# Autodesk Inventor assembly: New Box ARm
(part 2 of 2)
- Mate:204: Clamping_Shaft_Collar_-_1_2_Hex_ID_217-2737:1 ↔ Hex Shaft ARm:1
- Mate:205: Clamping_Shaft_Collar_-_1_2_Hex_ID_217-2737:1 ↔ Hex Shaft ARm:1
- Mate:213: 1_2_Acetal_Spacer_-_1_2_Hex_217-3261:1 ↔ Hex Shaft ARm:1
- Mate:214: 1_2_Acetal_Spacer_-_1_2_Hex_217-3261:1 ↔ Hex Shaft ARm:1
- Mate:215: 1_2_Acetal_Spacer_-_1_2_Hex_217-3261:1 ↔ 0_500_ID_x_1_125_OD_x_0_313_WD_Flanged_Bearing_217-2731:2
- Mate:222: 41.75in Arm Beam Alternate (Right):1 ↔ Hex Hub:2
- Mate:224: Hex Hub:2 ↔ Hex Shaft ARm:1
- Mate:225: Hex Hub:2 ↔ Hex Shaft ARm:1
- Mate:230: Hex Shaft ARm:1 ↔ 1_2_Acetal_Spacer_-_1_2_Hex_217-3261:4
- Mate:231: Hex Shaft ARm:1 ↔ 1_2_Acetal_Spacer_-_1_2_Hex_217-3261:4
- Mate:232: 1_2_Acetal_Spacer_-_1_2_Hex_217-3261:4 ↔ 0_500_ID_x_1_125_OD_x_0_313_WD_Flanged_Bearing_217-2731:3
- Mate:236: Hex Shaft ARm:1 ↔ Clamping_Shaft_Collar_-_1_2_Hex_ID_217-2737:2
- Mate:237: Hex Shaft ARm:1 ↔ Clamping_Shaft_Collar_-_1_2_Hex_ID_217-2737:2
- Mate:240: Hex Shaft ARm:1 ↔ Hex Hub:3
- Mate:241: Hex Shaft ARm:1 ↔ Hex Hub:3
- Rotation:2 [RelateRotation] (1 ul): Hex Shaft ARm:1 ↔ Hex Hub:3
- Rotation:4 [RelateRotation] (1 ul): Hex Hub:2 ↔ Hex Shaft ARm:1
- Mate:242: 15in Horizontal 1x1 Beam:1 ↔ 41.75in Arm Beam Alternate (Right):1
- Mate:259: L gusset:9 ↔ 1.5in 92196A251_18-8 STAINLESS STEEL SOCKET HEAD CAP SCREW:13
- Mate:260: L gusset:9 ↔ 1.5in 92196A251_18-8 STAINLESS STEEL SOCKET HEAD CAP SCREW:39
- Mate:261: L gusset:9 ↔ 1.5in 92196A251_18-8 STAINLESS STEEL SOCKET HEAD CAP SCREW:24
- Mate:263: L gusset:9 ↔ 1.5in 92196A251_18-8 STAINLESS STEEL SOCKET HEAD CAP SCREW:38
- Mate:268: L gusset:14 ↔ 1.5in 92196A251_18-8 STAINLESS STEEL SOCKET HEAD CAP SCREW:49
- Mate:269: L gusset:14 ↔ 1.5in 92196A251_18-8 STAINLESS STEEL SOCKET HEAD CAP SCREW:47
- Mate:270: L gusset:14 ↔ 1.5in 92196A251_18-8 STAINLESS STEEL SOCKET HEAD CAP SCREW:10
- Mate:271: L gusset:14 ↔ 1.5in 92196A251_18-8 STAINLESS STEEL SOCKET HEAD CAP SCREW:9
- Mate:272: L gusset:14 ↔ 1.5in 92196A251_18-8 STAINLESS STEEL SOCKET HEAD CAP SCREW:45
- Mate:273: L gusset:8 ↔ 1.5in 92196A251_18-8 STAINLESS STEEL SOCKET HEAD CAP SCREW:35
- Mate:274: L gusset:8 ↔ 1.5in 92196A251_18-8 STAINLESS STEEL SOCKET HEAD CAP SCREW:36
- Mate:275: L gusset:8 ↔ 1.5in 92196A251_18-8 STAINLESS STEEL SOCKET HEAD CAP SCREW:25
- Mate:277: L gusset:8 ↔ 1.5in 92196A251_18-8 STAINLESS STEEL SOCKET HEAD CAP SCREW:43
- Mate:278: L gusset:14 ↔ 1.5in 92196A251_18-8 STAINLESS STEEL SOCKET HEAD CAP SCREW:47
- Mate:279: L gusset:14 ↔ 1.5in 92196A251_18-8 STAINLESS STEEL SOCKET HEAD CAP SCREW:49
- Mate:280: L gusset:14 ↔ 1.5in 92196A251_18-8 STAINLESS STEEL SOCKET HEAD CAP SCREW:10
- Mate:281: L gusset:14 ↔ 1.5in 92196A251_18-8 STAINLESS STEEL SOCKET HEAD CAP SCREW:9
- Mate:282: L gusset:14 ↔ 1.5in 92196A251_18-8 STAINLESS STEEL SOCKET HEAD CAP SCREW:45
- Mate:285: L gusset:9 ↔ 1.5in 92196A251_18-8 STAINLESS STEEL SOCKET HEAD CAP SCREW:39
- Mate:286: L gusset:9 ↔ 1.5in 92196A251_18-8 STAINLESS STEEL SOCKET HEAD CAP SCREW:24
- Mate:287: L gusset:9 ↔ 1.5in 92196A251_18-8 STAINLESS STEEL SOCKET HEAD CAP SCREW:38
- Mate:288: L gusset:9 ↔ 1.5in 92196A251_18-8 STAINLESS STEEL SOCKET HEAD CAP SCREW:13
- Mate:289: L gusset:8 ↔ 1.5in 92196A251_18-8 STAINLESS STEEL SOCKET HEAD CAP SCREW:43
- Mate:291: L gusset:8 ↔ 1.5in 92196A251_18-8 STAINLESS STEEL SOCKET HEAD CAP SCREW:25
- Mate:292: L gusset:8 ↔ 1.5in 92196A251_18-8 STAINLESS STEEL SOCKET HEAD CAP SCREW:36
- Mate:293: L gusset:8 ↔ 1.5in 92196A251_18-8 STAINLESS STEEL SOCKET HEAD CAP SCREW:35
- Mate:296: L gusset:10 ↔ 1.5in 92196A251_18-8 STAINLESS STEEL SOCKET HEAD CAP SCREW:34
- Mate:297: L gusset:10 ↔ 1.5in 92196A251_18-8 STAINLESS STEEL SOCKET HEAD CAP SCREW:15
- Mate:298: L gusset:10 ↔ 1.5in 92196A251_18-8 STAINLESS STEEL SOCKET HEAD CAP SCREW:17
- Mate:300: 24in Vertical 1x1 Beam:3 ↔ LV Gusset:2
- Mate:301: 25in Horizontal 1x1 Beam:1 ↔ LV Gusset:2
- Mate:302: 25in Horizontal 1x1 Beam:1 ↔ LV Gusset:2
- Mate:303: 25in Horizontal 1x1 Beam:1 ↔ LV Gusset:2
- Mate:304: 24in Vertical 1x1 Beam:3 ↔ LV Gusset:2
- Mate:305: 24in Vertical 1x1 Beam:3 ↔ LV Gusset:2
- Mate:306: 24in Vertical 1x1 Beam:4 ↔ LV Gusset:1
- Mate:307: 25in Horizontal 1x1 Beam:2 ↔ LV Gusset:1
- Mate:308: 25in Horizontal 1x1 Beam:2 ↔ LV Gusset:1
- Mate:309: 25in Horizontal 1x1 Beam:2 ↔ LV Gusset:1
- Mate:310: 24in Vertical 1x1 Beam:4 ↔ LV Gusset:1
- Mate:311: 24in Vertical 1x1 Beam:4 ↔ LV Gusset:1
- Flush:129: 25in Horizontal 1x1 Beam:2 ↔ LV Gusset:1
- Flush:130: 24in Vertical 1x1 Beam:4 ↔ LV Gusset:1
- Flush:131: 24in Vertical 1x1 Beam:4 ↔ LV Gusset:1
- Flush:132: 25in Horizontal 1x1 Beam:2 ↔ LV Gusset:1
- Flush:133: 25in Horizontal 1x1 Beam:1 ↔ LV Gusset:2
- Flush:134: 24in Vertical 1x1 Beam:3 ↔ LV Gusset:2
- Flush:135: 24in Vertical 1x1 Beam:3 ↔ LV Gusset:2
- Flush:136: 25in Horizontal 1x1 Beam:1 ↔ LV Gusset:2
- Mate:312: 1.5in 92196A251_18-8 STAINLESS STEEL SOCKET HEAD CAP SCREW:7 ↔ LV Gusset:2
- Mate:313: 1.5in 92196A251_18-8 STAINLESS STEEL SOCKET HEAD CAP SCREW:11 ↔ LV Gusset:2
- Mate:314: 1.5in 92196A251_18-8 STAINLESS STEEL SOCKET HEAD CAP SCREW:11 ↔ LV Gusset:2
- Mate:315: 1.5in 92196A251_18-8 STAINLESS STEEL SOCKET HEAD CAP SCREW:7 ↔ LV Gusset:2
- Mate:316: 1.5in 92196A251_18-8 STAINLESS STEEL SOCKET HEAD CAP SCREW:14 ↔ LV Gusset:2
- Mate:317: 1.5in 92196A251_18-8 STAINLESS STEEL SOCKET HEAD CAP SCREW:2 ↔ LV Gusset:2
- Mate:318: 1.5in 92196A251_18-8 STAINLESS STEEL SOCKET HEAD CAP SCREW:14 ↔ LV Gusset:2
- Mate:319: 1.5in 92196A251_18-8 STAINLESS STEEL SOCKET HEAD CAP SCREW:2 ↔ LV Gusset:2
- Mate:320: 1.5in 92196A251_18-8 STAINLESS STEEL SOCKET HEAD CAP SCREW:1 ↔ LV Gusset:1
- Mate:321: 1.5in 92196A251_18-8 STAINLESS STEEL SOCKET HEAD CAP SCREW:20 ↔ LV Gusset:1
- Mate:322: 1.5in 92196A251_18-8 STAINLESS STEEL SOCKET HEAD CAP SCREW:1 ↔ LV Gusset:1
- Mate:323: 1.5in 92196A251_18-8 STAINLESS STEEL SOCKET HEAD CAP SCREW:20 ↔ LV Gusset:1
- Mate:324: 1.5in 92196A251_18-8 STAINLESS STEEL SOCKET HEAD CAP SCREW:3 ↔ LV Gusset:1
- Mate:325: 1.5in 92196A251_18-8 STAINLESS STEEL SOCKET HEAD CAP SCREW:8 ↔ LV Gusset:1
- Mate:326: 1.5in 92196A251_18-8 STAINLESS STEEL SOCKET HEAD CAP SCREW:8 ↔ LV Gusset:1
- Mate:327: 1.5in 92196A251_18-8 STAINLESS STEEL SOCKET HEAD CAP SCREW:3 ↔ LV Gusset:1
- Mate:328: L gusset:10 ↔ 1.5in 92196A251_18-8 STAINLESS STEEL SOCKET HEAD CAP SCREW:34
- Mate:329: L gusset:10 ↔ 1.5in 92196A251_18-8 STAINLESS STEEL SOCKET HEAD CAP SCREW:15
- Mate:330: L gusset:10 ↔ 1.5in 92196A251_18-8 STAINLESS STEEL SOCKET HEAD CAP SCREW:17
- Mate:332: L gusset:13 ↔ 1.5in 92196A251_18-8 STAINLESS STEEL SOCKET HEAD CAP SCREW:12
- Mate:333: L gusset:13 ↔ 1.5in 92196A251_18-8 STAINLESS STEEL SOCKET HEAD CAP SCREW:26
- Mate:334: L gusset:13 ↔ 1.5in 92196A251_18-8 STAINLESS STEEL SOCKET HEAD CAP SCREW:22
- Mate:335: L gusset:13 ↔ 1.5in 92196A251_18-8 STAINLESS STEEL SOCKET HEAD CAP SCREW:30
- Mate:336: L gusset:13 ↔ 1.5in 92196A251_18-8 STAINLESS STEEL SOCKET HEAD CAP SCREW:18
- Mate:337: L gusset:10 ↔ 1.5in 92196A251_18-8 STAINLESS STEEL SOCKET HEAD CAP SCREW:28
- Mate:338: L gusset:10 ↔ 1.5in 92196A251_18-8 STAINLESS STEEL SOCKET HEAD CAP SCREW:28
- Mate:339: L gusset:15 ↔ 1.5in 92196A251_18-8 STAINLESS STEEL SOCKET HEAD CAP SCREW:21
- Mate:340: L gusset:15 ↔ 1.5in 92196A251_18-8 STAINLESS STEEL SOCKET HEAD CAP SCREW:21
- Mate:341: L gusset:15 ↔ 1.5in 92196A251_18-8 STAINLESS STEEL SOCKET HEAD CAP SCREW:5
- Mate:342: L gusset:15 ↔ 1.5in 92196A251_18-8 STAINLESS STEEL SOCKET HEAD CAP SCREW:52
- Mate:343: L gusset:19 ↔ 1.5in 92196A251_18-8 STAINLESS STEEL SOCKET HEAD CAP SCREW:51
- Mate:344: L gusset:19 ↔ 1.5in 92196A251_18-8 STAINLESS STEEL SOCKET HEAD CAP SCREW:58
- Mate:345: L gusset:19 ↔ 1.5in 92196A251_18-8 STAINLESS STEEL SOCKET HEAD CAP SCREW:59
- Mate:346: L gusset:19 ↔ 1.5in 92196A251_18-8 STAINLESS STEEL SOCKET HEAD CAP SCREW:59
- Mate:347: L gusset:19 ↔ 1.5in 92196A251_18-8 STAINLESS STEEL SOCKET HEAD CAP SCREW:58
- Mate:348: L gusset:19 ↔ 1.5in 92196A251_18-8 STAINLESS STEEL SOCKET HEAD CAP SCREW:51
- Mate:349: L gusset:15 ↔ 1.5in 92196A251_18-8 STAINLESS STEEL SOCKET HEAD CAP SCREW:52
- Mate:350: L gusset:15 ↔ 1.5in 92196A251_18-8 STAINLESS STEEL SOCKET HEAD CAP SCREW:5
- Mate:351: L gusset:16 ↔ 1.5in 92196A251_18-8 STAINLESS STEEL SOCKET HEAD CAP SCREW:67
- Mate:352: L gusset:16 ↔ 1.5in 92196A251_18-8 STAINLESS STEEL SOCKET HEAD CAP SCREW:61
- Mate:353: L gusset:18 ↔ 1.5in 92196A251_18-8 STAINLESS STEEL SOCKET HEAD CAP SCREW:64
- Mate:354: L gusset:18 ↔ 1.5in 92196A251_18-8 STAINLESS STEEL SOCKET HEAD CAP SCREW:60
- Mate:355: L gusset:18 ↔ 1.5in 92196A251_18-8 STAINLESS STEEL SOCKET HEAD CAP SCREW:60
- Mate:356: L gusset:18 ↔ 1.5in 92196A251_18-8 STAINLESS STEEL SOCKET HEAD CAP SCREW:64
- Mate:357: L gusset:16 ↔ 1.5in 92196A251_18-8 STAINLESS STEEL SOCKET HEAD CAP SCREW:67
- Mate:358: L gusset:16 ↔ 1.5in 92196A251_18-8 STAINLESS STEEL SOCKET HEAD CAP SCREW:61
- Mate:359: L gusset:13 ↔ 1.5in 92196A251_18-8 STAINLESS STEEL SOCKET HEAD CAP SCREW:22
- Mate:360: L gusset:13 ↔ 1.5in 92196A251_18-8 STAINLESS STEEL SOCKET HEAD CAP SCREW:26
- Mate:361: L gusset:13 ↔ 1.5in 92196A251_18-8 STAINLESS STEEL SOCKET HEAD CAP SCREW:12
- Mate:362: L gusset:13 ↔ 1.5in 92196A251_18-8 STAINLESS STEEL SOCKET HEAD CAP SCREW:30
- Mate:363: L gusset:13 ↔ 1.5in 92196A251_18-8 STAINLESS STEEL SOCKET HEAD CAP SCREW:18
- Mate:364: L gusset:11 ↔ 1.5in 92196A251_18-8 STAINLESS STEEL SOCKET HEAD CAP SCREW:6
- Mate:365: L gusset:11 ↔ 1.5in 92196A251_18-8 STAINLESS STEEL SOCKET HEAD CAP SCREW:27
- Mate:366: L gusset:11 ↔ 1.5in 92196A251_18-8 STAINLESS STEEL SOCKET HEAD CAP SCREW:19
- Mate:368: L gusset:11 ↔ 1.5in 92196A251_18-8 STAINLESS STEEL SOCKET HEAD CAP SCREW:31
- Mate:369: L gusset:11 ↔ 1.5in 92196A251_18-8 STAINLESS STEEL SOCKET HEAD CAP SCREW:6
- Mate:370: L gusset:11 ↔ 1.5in 92196A251_18-8 STAINLESS STEEL SOCKET HEAD CAP SCREW:27
- Mate:372: L gusset:11 ↔ 1.5in 92196A251_18-8 STAINLESS STEEL SOCKET HEAD CAP SCREW:19
- Mate:373: L gusset:11 ↔ 1.5in 92196A251_18-8 STAINLESS STEEL SOCKET HEAD CAP SCREW:31
- Mate:376: L gusset:17 ↔ .75in 92196A245_18-8 STAINLESS STEEL SOCKET HEAD CAP SCREW:1
- Mate:377: L gusset:17 ↔ .75in 92196A245_18-8 STAINLESS STEEL SOCKET HEAD CAP SCREW:1
- Mate:380: L gusset:11 ↔ 1.5in 92196A251_18-8 STAINLESS STEEL SOCKET HEAD CAP SCREW:68
- Mate:381: L gusset:11 ↔ 1.5in 92196A251_18-8 STAINLESS STEEL SOCKET HEAD CAP SCREW:68
- Mate:382: L gusset:8 ↔ 1.5in 92196A251_18-8 STAINLESS STEEL SOCKET HEAD CAP SCREW:69
- Mate:383: L gusset:8 ↔ 1.5in 92196A251_18-8 STAINLESS STEEL SOCKET HEAD CAP SCREW:69
- Mate:384: L gusset:20 ↔ .75in 92196A245_18-8 STAINLESS STEEL SOCKET HEAD CAP SCREW:34
- Mate:385: L gusset:20 ↔ .75in 92196A245_18-8 STAINLESS STEEL SOCKET HEAD CAP SCREW:34
- Mate:386: L gusset:20 ↔ .75in 92196A245_18-8 STAINLESS STEEL SOCKET HEAD CAP SCREW:14
- Mate:387: L gusset:20 ↔ .75in 92196A245_18-8 STAINLESS STEEL SOCKET HEAD CAP SCREW:15
- Mate:388: L gusset:17 ↔ .75in 92196A245_18-8 STAINLESS STEEL SOCKET HEAD CAP SCREW:17
- Mate:389: L gusset:17 ↔ .75in 92196A245_18-8 STAINLESS STEEL SOCKET HEAD CAP SCREW:58
- Mate:390: L gusset:17 ↔ .75in 92196A245_18-8 STAINLESS STEEL SOCKET HEAD CAP SCREW:17
- Mate:391: L gusset:17 ↔ .75in 92196A245_18-8 STAINLESS STEEL SOCKET HEAD CAP SCREW:58
- Mate:392: L gusset:20 ↔ .75in 92196A245_18-8 STAINLESS STEEL SOCKET HEAD CAP SCREW:14
- Mate:393: L gusset:20 ↔ .75in 92196A245_18-8 STAINLESS STEEL SOCKET HEAD CAP SCREW:15
- Mate:394: L gusset:17 ↔ 1.5in 92196A251_18-8 STAINLESS STEEL SOCKET HEAD CAP SCREW:54
- Mate:395: L gusset:17 ↔ 1.5in 92196A251_18-8 STAINLESS STEEL SOCKET HEAD CAP SCREW:33
- Mate:396: L gusset:20 ↔ 1.5in 92196A251_18-8 STAINLESS STEEL SOCKET HEAD CAP SCREW:56
- Mate:397: L gusset:20 ↔ 1.5in 92196A251_18-8 STAINLESS STEEL SOCKET HEAD CAP SCREW:50
- Mate:398: L gusset:20 ↔ 1.5in 92196A251_18-8 STAINLESS STEEL SOCKET HEAD CAP SCREW:56
- Mate:399: L gusset:20 ↔ 1.5in 92196A251_18-8 STAINLESS STEEL SOCKET HEAD CAP SCREW:50
- Mate:400: L gusset:17 ↔ 1.5in 92196A251_18-8 STAINLESS STEEL SOCKET HEAD CAP SCREW:54
- Mate:401: L gusset:17 ↔ 1.5in 92196A251_18-8 STAINLESS STEEL SOCKET HEAD CAP SCREW:33
- Mate:403: 41.75in Arm Beam Alternate (Right):1 ↔ 0_500_ID_x_1_125_OD_x_0_313_WD_Flanged_Bearing_217-2731:6
- Mate:404: 41.75in Arm Beam Alternate (Right):1 ↔ 0_500_ID_x_1_125_OD_x_0_313_WD_Flanged_Bearing_217-2731:7
- Mate:409: 41.75in Arm Beam Alternate (Right):1 ↔ 0_500_ID_x_1_125_OD_x_0_313_WD_Flanged_Bearing_217-2731:6
- Mate:410: 41.75in Arm Beam Alternate (Right):1 ↔ 0_500_ID_x_1_125_OD_x_0_313_WD_Flanged_Bearing_217-2731:7
- Mate:411: 41.75in Arm Beam Alternate (Right):1 ↔ 0_500_Hex_ID_x_1_125_OD_x_0_313_WD_Flanged_Bearing_v2_217-3875:1
- Mate:418: 41.75in Arm Beam Alternate (Right):1 ↔ 0_500_Hex_ID_x_1_125_OD_x_0_313_WD_Flanged_Bearing_v2_217-3875:1
- Mate:419: 41.75in Arm Beam Alternate (Right):1 ↔ VersaPlanetary_v2_Two_Stage_100_1_with_BAG:1
- Mate:420: 41.75in Arm Beam Alternate (Right):1 ↔ VersaPlanetary_v2_Two_Stage_100_1_with_BAG:1
- Mate:421: 41.75in Arm Beam Alternate (Right):1 ↔ VersaPlanetary_v2_Two_Stage_100_1_with_BAG:1
- Mate:422: am-3621 - S25-18HA-500H:1 ↔ VersaPlanetary_v2_Two_Stage_100_1_with_BAG:1
- Mate:423: am-3621 - S25-18HA-500H:1 ↔ VersaPlanetary_v2_Two_Stage_100_1_with_BAG:1
- Mate:424: am-3621 - S25-18HA-500H:1 ↔ 0_500_Hex_ID_x_1_125_OD_x_0_313_WD_Flanged_Bearing_v2_217-3875:1
- Mate:426: VersaPlanetary_v2_Two_Stage_100_1_with_BAG:1 ↔ 3D Model Spacer Arm:1
- Mate:427: VersaPlanetary_v2_Two_Stage_100_1_with_BAG:1 ↔ 3D Model Spacer Arm:1
- Mate:428: am-3621 - S25-18HA-500H:1 ↔ 3D Model Spacer Arm:1
- Mate:429: VersaPlanetary_v2_Two_Stage_100_1_with_BAG:1 ↔ 92240A537_18-8 STAINLESS STEEL HEX HEAD CAP SCREW:1
- Mate:430: 92240A537_18-8 STAINLESS STEEL HEX HEAD CAP SCREW:1 ↔ 3D Model Washer Arm Gearbo:1
- Mate:431: 3D Model Spacer Arm:1 ↔ 3D Model Washer Arm Gearbo:1
- Mate:432: 92240A537_18-8 STAINLESS STEEL HEX HEAD CAP SCREW:1 ↔ 3D Model Washer Arm Gearbo:1
- Mate:437: Wrist Hex Shaft 0.5in:1 ↔ Clamping_Shaft_Collar_-_1_2_Hex_ID_217-2737:6
- Mate:438: Wrist Hex Shaft 0.5in:1 ↔ Clamping_Shaft_Collar_-_1_2_Hex_ID_217-2737:6
- Flush:138: Wrist Hex Shaft 0.5in:1 ↔ Clamping_Shaft_Collar_-_1_2_Hex_ID_217-2737:6
- Mate:439: Wrist Hex Shaft 0.5in:1 ↔ Clamping_Shaft_Collar_-_1_2_Hex_ID_217-2737:5
- Mate:440: Wrist Hex Shaft 0.5in:1 ↔ Clamping_Shaft_Collar_-_1_2_Hex_ID_217-2737:5
- Mate:441: Wrist Hex Shaft 0.5in:1 ↔ Clamping_Shaft_Collar_-_1_2_Hex_ID_217-2737:4
- Mate:442: Wrist Hex Shaft 0.5in:1 ↔ Clamping_Shaft_Collar_-_1_2_Hex_ID_217-2737:4
- Mate:443: Wrist Hex Shaft 0.5in:1 ↔ 1_16_Acetal_Spacer_-_1_2_Hex_217-3257:2
- Mate:444: Wrist Hex Shaft 0.5in:1 ↔ 1_16_Acetal_Spacer_-_1_2_Hex_217-3257:2
- Mate:445: Wrist Hex Shaft 0.5in:1 ↔ 1_16_Acetal_Spacer_-_1_2_Hex_217-3257:1
- Mate:446: Wrist Hex Shaft 0.5in:1 ↔ 1_16_Acetal_Spacer_-_1_2_Hex_217-3257:1
- Mate:447: 0_500_ID_x_1_125_OD_x_0_313_WD_Flanged_Bearing_217-2731:6 ↔ 1_16_Acetal_Spacer_-_1_2_Hex_217-3257:1
- Mate:448: Clamping_Shaft_Collar_-_1_2_Hex_ID_217-2737:4 ↔ 1_16_Acetal_Spacer_-_1_2_Hex_217-3257:1
- Mate:449: 0_500_ID_x_1_125_OD_x_0_313_WD_Flanged_Bearing_217-2731:5 ↔ 1_16_Acetal_Spacer_-_1_2_Hex_217-3257:2
- Mate:450: Clamping_Shaft_Collar_-_1_2_Hex_ID_217-2737:5 ↔ 1_16_Acetal_Spacer_-_1_2_Hex_217-3257:2
- Mate:451: am-3621 - S25-18HA-500H:2 ↔ Wrist Hex Shaft 0.5in:1
- Mate:452: am-3621 - S25-18HA-500H:2 ↔ Wrist Hex Shaft 0.5in:1
- Mate:453: 0_500_ID_x_1_125_OD_x_0_313_WD_Flanged_Bearing_217-2731:7 ↔ am-3621 - S25-18HA-500H:2
- Flush:140: am-3621 - S25-18HA-500H:1 ↔ am-3621 - S25-18HA-500H:2
- Mate:459: 0_500_ID_x_1_125_OD_x_0_313_WD_Flanged_Bearing_217-2731:6 ↔ 1_16_Acetal_Spacer_-_1_2_Hex_217-3257:1
- Mate:460: 0_500_ID_x_1_125_OD_x_0_313_WD_Flanged_Bearing_217-2731:8 ↔ Clamping_Shaft_Collar_-_1_2_Hex_ID_217-2737:6
- Mate:482: Hex Hub:3 ↔ 41.75in Arm Beam Alternate (Left):1
- Mate:488: Hex Hub:3 ↔ 41.75in Arm Beam Alternate (Left):1
- Mate:489: 0_500_ID_x_1_125_OD_x_0_313_WD_Flanged_Bearing_217-2731:10 ↔ 41.75in Arm Beam Alternate (Left):1
- Mate:490: 0_500_ID_x_1_125_OD_x_0_313_WD_Flanged_Bearing_217-2731:10 ↔ 41.75in Arm Beam Alternate (Left):1
- Mate:491: 41.75in Arm Beam Alternate (Right):1 ↔ 0_500_ID_x_1_125_OD_x_0_313_WD_Flanged_Bearing_217-2731:9
- Mate:492: 41.75in Arm Beam Alternate (Right):1 ↔ 0_500_ID_x_1_125_OD_x_0_313_WD_Flanged_Bearing_217-2731:9
- Mate:493: 0_500_ID_x_1_125_OD_x_0_313_WD_Flanged_Bearing_217-2731:8 ↔ Clamping_Shaft_Collar_-_1_2_Hex_ID_217-2737:6
- Mate:494: 0_500_ID_x_1_125_OD_x_0_313_WD_Flanged_Bearing_217-2731:5 ↔ 41.75in Arm Beam Alternate (Left):1
- Mate:495: 0_500_ID_x_1_125_OD_x_0_313_WD_Flanged_Bearing_217-2731:5 ↔ 41.75in Arm Beam Alternate (Left):1
- Mate:506: 15in Horizontal 1x1 Beam:2 ↔ 1x1 Bumper Attachment:2
- Mate:507: 15in Horizontal 1x1 Beam:2 ↔ 1x1 Bumper Attachment:2
- Mate:508: 15in Horizontal 1x1 Beam:2 ↔ 1x1 Bumper Attachment:2
- Mate:509: 15in Horizontal 1x1 Beam:1 ↔ 1x1 Bumper Attachment:1
- Mate:510: 15in Horizontal 1x1 Beam:1 ↔ 1x1 Bumper Attachment:1
- Mate:511: 15in Horizontal 1x1 Beam:1 ↔ 1x1 Bumper Attachment:1
- Mate:512: 1x1 Bumper Attachment:2 ↔ 042:1
- Mate:513: 1x1 Bumper Attachment:2 ↔ 042:1
- Mate:514: 1x1 Bumper Attachment:1 ↔ 042:2
- Mate:515: 1x1 Bumper Attachment:1 ↔ 042:2
- Mate:516: 15in Horizontal 1x1 Beam:1 ↔ Arm Belly Pan:1
- Mate:517: L gusset:1 ↔ Arm Belly Pan:1
- Flush:141: 15in Horizontal 1x1 Beam:1 ↔ Arm Belly Pan:1
- Mate:518: Hex Hub:3 ↔ 41.75in Arm Beam Alternate (Left):1
- Mate:519: Hex Hub:3 ↔ 41.75in Arm Beam Alternate (Left):1
- Mate:522: Arm Belly Pan:1 ↔ 73434-Fastenal-01-12-2019:2
- Mate:523: Arm Belly Pan:1 ↔ 73434-Fastenal-01-12-2019:1
- Mate:524: Arm Belly Pan:1 ↔ 73434-Fastenal-01-12-2019:2
- Mate:525: Arm Belly Pan:1 ↔ 73434-Fastenal-01-12-2019:1
- Mate:526: Arm Belly Pan:1 ↔ 73434-Fastenal-01-12-2019:4
- Mate:527: Arm Belly Pan:1 ↔ 73434-Fastenal-01-12-2019:3
- Mate:528: Arm Belly Pan:1 ↔ 73434-Fastenal-01-12-2019:3
- Mate:529: Arm Belly Pan:1 ↔ 73434-Fastenal-01-12-2019:4
- Mate:530: 1x1 Bumper Attachment:1 ↔ 91831A011_TYPE 18-8 STAINLESS STL NYLON-INSERT LOCKNUT:4
- Mate:531: 73434-Fastenal-01-12-2019:3 ↔ 91831A011_TYPE 18-8 STAINLESS STL NYLON-INSERT LOCKNUT:4
- Mate:532: 1x1 Bumper Attachment:1 ↔ 91831A011_TYPE 18-8 STAINLESS STL NYLON-INSERT LOCKNUT:3
- Mate:533: 73434-Fastenal-01-12-2019:4 ↔ 91831A011_TYPE 18-8 STAINLESS STL NYLON-INSERT LOCKNUT:3
- Mate:534: 1x1 Bumper Attachment:2 ↔ 91831A011_TYPE 18-8 STAINLESS STL NYLON-INSERT LOCKNUT:2
- Mate:535: 73434-Fastenal-01-12-2019:1 ↔ 91831A011_TYPE 18-8 STAINLESS STL NYLON-INSERT LOCKNUT:2
- Mate:536: 1x1 Bumper Attachment:2 ↔ 91831A011_TYPE 18-8 STAINLESS STL NYLON-INSERT LOCKNUT:1
- Mate:537: 73434-Fastenal-01-12-2019:2 ↔ 91831A011_TYPE 18-8 STAINLESS STL NYLON-INSERT LOCKNUT:1
- Mate:538: Arm Belly Pan:1 ↔ 1.5in 92196A251_18-8 STAINLESS STEEL SOCKET HEAD CAP SCREW:73
- Mate:539: Arm Belly Pan:1 ↔ 1.5in 92196A251_18-8 STAINLESS STEEL SOCKET HEAD CAP SCREW:72
- Mate:540: Arm Belly Pan:1 ↔ 1.5in 92196A251_18-8 STAINLESS STEEL SOCKET HEAD CAP SCREW:70
- Mate:541: Arm Belly Pan:1 ↔ 1.5in 92196A251_18-8 STAINLESS STEEL SOCKET HEAD CAP SCREW:71
- Mate:542: Arm Belly Pan:1 ↔ 73434-Fastenal-01-12-2019:6
- Mate:543: Arm Belly Pan:1 ↔ 73434-Fastenal-01-12-2019:5
- Mate:544: Arm Belly Pan:1 ↔ 73434-Fastenal-01-12-2019:8
- Mate:545: Arm Belly Pan:1 ↔ 73434-Fastenal-01-12-2019:7
- Mate:546 (3.175 mm): Arm Belly Pan:1 ↔ 73434-Fastenal-01-12-2019:7
- Mate:547 (3.175 mm): Arm Belly Pan:1 ↔ 73434-Fastenal-01-12-2019:8
- Mate:548 (3.175 mm): Arm Belly Pan:1 ↔ 1.5in 92196A251_18-8 STAINLESS STEEL SOCKET HEAD CAP SCREW:73
- Mate:549 (3.175 mm): Arm Belly Pan:1 ↔ 1.5in 92196A251_18-8 STAINLESS STEEL SOCKET HEAD CAP SCREW:72
- Mate:550 (3.175 mm): Arm Belly Pan:1 ↔ 1.5in 92196A251_18-8 STAINLESS STEEL SOCKET HEAD CAP SCREW:70
- Mate:551 (3.175 mm): Arm Belly Pan:1 ↔ 1.5in 92196A251_18-8 STAINLESS STEEL SOCKET HEAD CAP SCREW:71
- Mate:552 (3.175 mm): Arm Belly Pan:1 ↔ 73434-Fastenal-01-12-2019:6
- Mate:553 (3.175 mm): Arm Belly Pan:1 ↔ 73434-Fastenal-01-12-2019:5
- Mate:554: 25in Horizontal 1x1 Beam:2 ↔ 91831A011_TYPE 18-8 STAINLESS STL NYLON-INSERT LOCKNUT:6
- Mate:555: 25in Horizontal 1x1 Beam:2 ↔ 91831A011_TYPE 18-8 STAINLESS STL NYLON-INSERT LOCKNUT:12
- Mate:556: Arm Belly Pan:1 ↔ 91831A011_TYPE 18-8 STAINLESS STL NYLON-INSERT LOCKNUT:5
- Mate:557: Arm Belly Pan:1 ↔ 91831A011_TYPE 18-8 STAINLESS STL NYLON-INSERT LOCKNUT:11
- Mate:558: Arm Belly Pan:1 ↔ 91831A011_TYPE 18-8 STAINLESS STL NYLON-INSERT LOCKNUT:8
- Mate:559: Arm Belly Pan:1 ↔ 91831A011_TYPE 18-8 STAINLESS STL NYLON-INSERT LOCKNUT:7
- Mate:560: 25in Horizontal 1x1 Beam:1 ↔ 91831A011_TYPE 18-8 STAINLESS STL NYLON-INSERT LOCKNUT:9
- Mate:561: 25in Horizontal 1x1 Beam:1 ↔ 91831A011_TYPE 18-8 STAINLESS STL NYLON-INSERT LOCKNUT:10
- Mate:562: 91831A011_TYPE 18-8 STAINLESS STL NYLON-INSERT LOCKNUT:10 ↔ 73434-Fastenal-01-12-2019:7
- Mate:563: 91831A011_TYPE 18-8 STAINLESS STL NYLON-INSERT LOCKNUT:9 ↔ 73434-Fastenal-01-12-2019:8
- Mate:564: 91831A011_TYPE 18-8 STAINLESS STL NYLON-INSERT LOCKNUT:7 ↔ 1.5in 92196A251_18-8 STAINLESS STEEL SOCKET HEAD CAP SCREW:73
- Mate:565: 91831A011_TYPE 18-8 STAINLESS STL NYLON-INSERT LOCKNUT:8 ↔ 1.5in 92196A251_18-8 STAINLESS STEEL SOCKET HEAD CAP SCREW:72
- Mate:566: 91831A011_TYPE 18-8 STAINLESS STL NYLON-INSERT LOCKNUT:5 ↔ 1.5in 92196A251_18-8 STAINLESS STEEL SOCKET HEAD CAP SCREW:70
- Mate:567: 91831A011_TYPE 18-8 STAINLESS STL NYLON-INSERT LOCKNUT:11 ↔ 1.5in 92196A251_18-8 STAINLESS STEEL SOCKET HEAD CAP SCREW:71
- Mate:568: 91831A011_TYPE 18-8 STAINLESS STL NYLON-INSERT LOCKNUT:12 ↔ 73434-Fastenal-01-12-2019:5
- Mate:569: 91831A011_TYPE 18-8 STAINLESS STL NYLON-INSERT LOCKNUT:6 ↔ 73434-Fastenal-01-12-2019:6
- Mate:575: ARm Gearbox:1 ↔ 0_500_ID_x_1_125_OD_x_0_313_WD_Flanged_Bearing_217-2731:12
- Mate:576: ARm Gearbox:1 ↔ 0_500_ID_x_1_125_OD_x_0_313_WD_Flanged_Bearing_217-2731:12
- Mate:577: Gearbox Shaft Stabilizer:1 ↔ 0_500_ID_x_1_125_OD_x_0_313_WD_Flanged_Bearing_217-2731:11
- Mate:578: Gearbox Shaft Stabilizer:1 ↔ 0_500_ID_x_1_125_OD_x_0_313_WD_Flanged_Bearing_217-2731:11
- Mate:579: Gearbox Shaft Stabilizer:1 ↔ 0_500_ID_x_1_125_OD_x_0_313_WD_Flanged_Bearing_217-2731:12
- Mate:580: Gearbox Shaft Stabilizer:1 ↔ 0_500_ID_x_1_125_OD_x_0_313_WD_Flanged_Bearing_217-2731:12
- Angle:1 (90 deg): Arm Belly Pan:1 ↔ Gearbox Shaft Stabilizer:1
- Mate:581: ARm Gearbox:1 ↔ Clamping_Shaft_Collar_-_1_2_Hex_ID_217-2737:8
- Mate:582: ARm Gearbox:1 ↔ Clamping_Shaft_Collar_-_1_2_Hex_ID_217-2737:8
- Mate:583: 0_500_ID_x_1_125_OD_x_0_313_WD_Flanged_Bearing_217-2731:11 ↔ Clamping_Shaft_Collar_-_1_2_Hex_ID_217-2737:8
- Mate:584: Gearbox Shaft Stabilizer:1 ↔ 1x2 L Bracket:1
- Mate:585: Gearbox Shaft Stabilizer:1 ↔ 1x2 L Bracket:1
- Mate:586: Gearbox Shaft Stabilizer:1 ↔ 1x2 L Bracket:1
- Mate:587: Gearbox Shaft Stabilizer:1 ↔ 1x2 L Bracket:1
- Mate:588: Gearbox Shaft Stabilizer:1 ↔ 1x2 L Bracket:2
- Mate:589: Gearbox Shaft Stabilizer:1 ↔ 1x2 L Bracket:2
- Mate:590: Gearbox Shaft Stabilizer:1 ↔ 1x2 L Bracket:2
- Mate:591: Gearbox Shaft Stabilizer:1 ↔ 1x2 L Bracket:2
- Flush:142: 41.75in Arm Beam Alternate (Right):1 ↔ non integrated hatch:1
- Flush:143: Wrist Hex Shaft 0.5in:1 ↔ non integrated hatch:1
- Mate:600: 41.75in Arm Beam Alternate (Left):1 ↔ non integrated hatch:1
- Mate:601: 0_500_ID_x_1_125_OD_x_0_313_WD_Flanged_Bearing_217-2731:12 ↔ Gearbox Shaft Stabilizer:2
- Mate:602: 0_500_ID_x_1_125_OD_x_0_313_WD_Flanged_Bearing_217-2731:11 ↔ Gearbox Shaft Stabilizer:2
- Mate:603: 0_500_ID_x_1_125_OD_x_0_313_WD_Flanged_Bearing_217-2731:11 ↔ Gearbox Shaft Stabilizer:2
- Mate:604: 0_500_ID_x_1_125_OD_x_0_313_WD_Flanged_Bearing_217-2731:12 ↔ Gearbox Shaft Stabilizer:2
- Angle:2 (90 deg): Arm Belly Pan:1 ↔ Gearbox Shaft Stabilizer:2
- Mate:608: Gearbox Shaft Stabilizer:2 ↔ 1x2 L Bracket:3
- Mate:609: Gearbox Shaft Stabilizer:2 ↔ 1x2 L Bracket:3
- Mate:610: Gearbox Shaft Stabilizer:2 ↔ 1x2 L Bracket:3
- Mate:611: Gearbox Shaft Stabilizer:2 ↔ 1x2 L Bracket:4
- Mate:612: Gearbox Shaft Stabilizer:2 ↔ 1x2 L Bracket:4
- Mate:613: Gearbox Shaft Stabilizer:2 ↔ 1x2 L Bracket:4
- Mate:614: 1x2 L Bracket:3 ↔ 1.5in 92196A251_18-8 STAINLESS STEEL SOCKET HEAD CAP SCREW:79
- Mate:615: 1x2 L Bracket:3 ↔ 1.5in 92196A251_18-8 STAINLESS STEEL SOCKET HEAD CAP SCREW:78
- Mate:616: 1x2 L Bracket:3 ↔ 1.5in 92196A251_18-8 STAINLESS STEEL SOCKET HEAD CAP SCREW:78
- Mate:617: 1x2 L Bracket:3 ↔ 1.5in 92196A251_18-8 STAINLESS STEEL SOCKET HEAD CAP SCREW:79
- Mate:621: _72t_Aluminum_Plate_Sprocket_25_Chain_1-1_8_Bearing_Bore_217-2627:1 ↔ Hex Hub:2
- Mate:622: _72t_Aluminum_Plate_Sprocket_25_Chain_1-1_8_Bearing_Bore_217-2627:1 ↔ Hex Hub:2
- Mate:623 (7.62 mm): _72t_Aluminum_Plate_Sprocket_25_Chain_1-1_8_Bearing_Bore_217-2627:1 ↔ 41.75in Arm Beam Alternate (Right):1
- Mate:624: _72t_Aluminum_Plate_Sprocket_25_Chain_1-1_8_Bearing_Bore_217-2627:1 ↔ Hex Hub:2
- Mate:625: _72t_Aluminum_Plate_Sprocket_25_Chain_1-1_8_Bearing_Bore_217-2627:1 ↔ Hex Hub:2
- Mate:631: Hex Shaft ARm:1 ↔ 1_2_Acetal_Spacer_-_1_2_Hex_217-3261:8
- Mate:632: Hex Shaft ARm:1 ↔ 1_2_Acetal_Spacer_-_1_2_Hex_217-3261:8
- Mate:633: 1_2_Acetal_Spacer_-_1_2_Hex_217-3261:1 ↔ 1_2_Acetal_Spacer_-_1_2_Hex_217-3261:8
- Mate:634: Hex Hub:2 ↔ 1_2_Acetal_Spacer_-_1_2_Hex_217-3261:8
- Mate:635: Hex Shaft ARm:1 ↔ 1_2_Acetal_Spacer_-_1_2_Hex_217-3261:10
- Mate:636: Hex Shaft ARm:1 ↔ 1_2_Acetal_Spacer_-_1_2_Hex_217-3261:10
- Mate:638: 1_2_Acetal_Spacer_-_1_2_Hex_217-3261:4 ↔ 1_2_Acetal_Spacer_-_1_2_Hex_217-3261:10
- Mate:639: Hex Hub:3 ↔ 1_2_Acetal_Spacer_-_1_2_Hex_217-3261:10
- Mate:640: Clamping_Shaft_Collar_-_1_2_Hex_ID_217-2737:2 ↔ 0_500_ID_x_1_125_OD_x_0_313_WD_Flanged_Bearing_217-2731:10
- Mate:641: Clamping_Shaft_Collar_-_1_2_Hex_ID_217-2737:1 ↔ 0_500_ID_x_1_125_OD_x_0_313_WD_Flanged_Bearing_217-2731:9
- Flush:144 (-25.4 mm): 30in Vertical 1x2 Beam:2 ↔ Hex Shaft ARm:1
- Mate:642: 41.75in Arm Beam Alternate (Right):1 ↔ Hard Stop:1
- Mate:644: 41.75in Arm Beam Alternate (Left):1 ↔ Hard Stop:1
